# Autodesk Inventor assembly: motor=sprocket
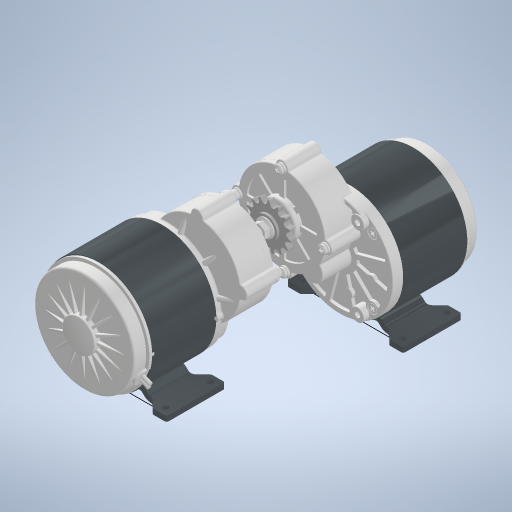
[picture p0: Inventor's stored thumbnail of the model, 512x512]
Saved by Autodesk Inventor 2023 (Build 270158000, 158)
## iProperties
Created: 2023-09-03
Part Number: motor=sprocket
Document SubType Name: Assembly
Designer: sigit
Author: sigit
## Documents named in this file (2)
- D:\Kuliah\SEMESTER 7\Robot Semprot\Design\REVISI2\Part\motor=sprocket.iam
- D:\Kuliah\SEMESTER 7\Robot Semprot\Design\REVISI2\Assembly\Motor DC - MY1016Z.iam
## Components (2 placed, 1 different names)
1. Motor DC - MY1016Z:1 [sub-assembly] — Rotational:1
2. Motor DC - MY1016Z:2 [sub-assembly] — Rotational:1
## Relationships (1: RevoluteJoint 1)
- Rotational:1 [RevoluteJoint]: Motor DC - MY1016Z:1 ↔ Motor DC - MY1016Z:2
